# Autodesk Inventor assembly: Sestava2
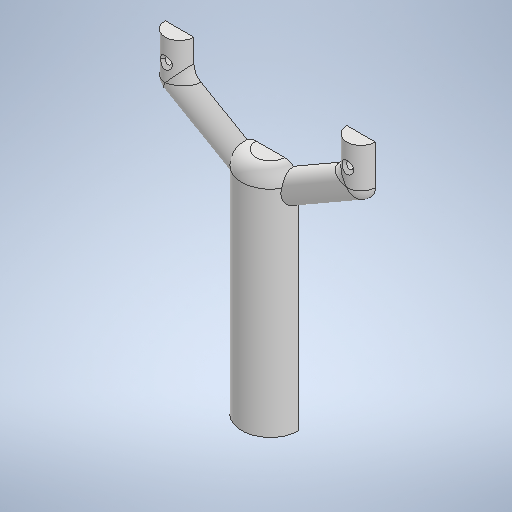
[picture p0: Inventor's stored thumbnail of the model, 512x512]
Saved by Autodesk Inventor 2025.2 (Build 292293000, 293)
## iProperties
Created: 2025-03-25
Part Number: Sestava2
Document SubType Name: Assembly
Designer: hepma_axt67em
Author: hepma_axt67em
## Documents named in this file (3)
- C:\Users\hepma_axt67em\Documents\Inventor\GeigerCounter\Sestava2.iam
- C:\Users\hepma_axt67em\Documents\Inventor\GeigerCounter\probe_1.ipt
- C:\Users\hepma_axt67em\Documents\Inventor\GeigerCounter\probe_2.ipt
## Components (2 placed, 2 different names)
1. probe_1:1 — Proti sobě:1, Stejný směr:1, Proti sobě:2
2. probe_2:1 — Proti sobě:1, Stejný směr:1, Proti sobě:2
## Relationships (3: Mate 2, Flush 1)
- Proti sobě:1 [Mate]: probe_1:1 ↔ probe_2:1
- Stejný směr:1 [Flush]: probe_1:1 ↔ probe_2:1
- Proti sobě:2 [Mate]: probe_1:1 ↔ probe_2:1
